# Autodesk Inventor assembly: Arm
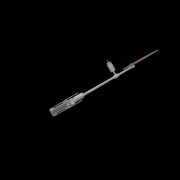
[picture p0: Inventor's stored thumbnail of the model, 180x180]
Saved by Autodesk Inventor 2020 (Build 240168000, 168)
## iProperties
Created: 2020-03-24
Part Number: Arm
Document SubType Name: Assembly
Designer: valer
Mass: 4853.44 g
Surface Area: 23913.7 cm^2
Volume: 23972.4 cm^3
Density: 0.202459 g/cm^3
Author: valer
## Documents named in this file (17)
- C:\Users\valer\Desktop\drummingrobot\src\Arm.iam
- C:\Users\valer\Desktop\drummingrobot\src\UpperArm.ipt
- C:\Users\valer\Desktop\drummingrobot\src\UpperArmBracket.ipt
- C:\Users\valer\Desktop\drummingrobot\src\Forearm.ipt
- C:\Users\valer\Desktop\drummingrobot\src\external\Drumstick.ipt
- C:\Users\valer\Desktop\drummingrobot\src\external\ForearmShaftCollar.ipt
- C:\Users\valer\Desktop\drummingrobot\src\external\PushSolenoid.ipt
- C:\Users\valer\Desktop\drummingrobot\src\external\UpperArmActuatorBody.ipt
- C:\Users\valer\Desktop\drummingrobot\src\external\UpperArmActuatorShaft.ipt
- C:\Users\valer\Desktop\drummingrobot\src\external\ForearmActuatorBody.ipt
- C:\Users\valer\Desktop\drummingrobot\src\external\ForearmActuatorShaft.ipt
- C:\Users\valer\Desktop\drummingrobot\src\external\Drums.ipt
- C:\Users\valer\Desktop\drummingrobot\src\ForearmActuatorConnector.ipt
- C:\Users\valer\Desktop\drummingrobot\src\UpperArmBracketMirror.ipt
- C:\Users\valer\Desktop\drummingrobot\src\UpperArmActuatorBracket.ipt
- C:\Users\valer\Desktop\drummingrobot\src\UpperArmActuatorBracketMirror.ipt
- C:\Users\valer\Desktop\drummingrobot\src\UpperArmMount.ipt
## Components (17 placed, 15 different names)
1. Drumstick:1 — Mate:79, Flush:3
2. ShaftCollar1/2:1 — Mate:79, Flush:3, Mate:236, Flush:18
3. PushSolenoid:1 — Mate:258, Mate:259
4. FA-35-S-12-1:1 — Mate:257, Mate:266
5. Forearm:1 — Flush:17, Mate:227, Mate:236, Flush:18, Mate:239, Mate:244, Mate:258, Mate:259
6. FA-35-S-12-1:2 — Mate:238, Flush:20, Mate:266
7. ForearmActuatorBody:1 — Mate:231, Mate:232, Mate:234, Flush:19
8. Drums:1 — Flush:13
9. ForearmActuatorShaft:3 — Flush:17, Mate:231, Mate:232, Mate:241, Mate:243, Angle:10, Mate:246
10. UpperArm:3 — Mate:227, Mate:234, Mate:238, Flush:19, Flush:20, Mate:248, Mate:249, Mate:263, Mate:264, Mate:265
11. ForearmActuatorConnector:1 — Mate:239, Mate:241, Mate:245, Angle:10, Mate:246
12. ForearmActuatorConnector:2 — Mate:243, Mate:244, Mate:245
13. UpperArmBracket:5 — Mate:249, Mate:254, Mate:255, Mate:256, Flush:21, Mate:265, Mate:267, Mate:272
14. UpperArmBracketMirror:1 — Mate:248, Mate:251, Mate:252, Mate:253, Flush:21, Mate:263, Mate:264, Mate:270, Mate:271
15. UpperArmActuatorBracket:1 — Mate:254, Mate:255, Mate:256, Mate:262
16. UpperArmActuatorBracketMirror:1 — Mate:251, Mate:252, Mate:253, Mate:257
17. UpperArmMount:1 — Mate:267, Mate:270, Mate:271, Mate:272, Mate:273
## Relationships (42: Mate 34, Flush 7, Angle 1)
- Mate:79: Drumstick:1 ↔ ShaftCollar1/2:1
- Flush:3 (304.8 mm): Drumstick:1 ↔ ShaftCollar1/2:1
- Flush:13 (508 mm): Drums:1
- Flush:17: Forearm:1 ↔ ForearmActuatorShaft:3
- Mate:227: Forearm:1 ↔ UpperArm:3
- Mate:231: ForearmActuatorBody:1 ↔ ForearmActuatorShaft:3
- Mate:232: ForearmActuatorBody:1 ↔ ForearmActuatorShaft:3
- Mate:234: ForearmActuatorBody:1 ↔ UpperArm:3
- Mate:236: ShaftCollar1/2:1 ↔ Forearm:1
- Flush:18 (12.7 mm): ShaftCollar1/2:1 ↔ Forearm:1
- Mate:238: FA-35-S-12-1:2 ↔ UpperArm:3
- Flush:19: ForearmActuatorBody:1 ↔ UpperArm:3
- Flush:20: FA-35-S-12-1:2 ↔ UpperArm:3
- Mate:239: Forearm:1 ↔ ForearmActuatorConnector:1
- Mate:241: ForearmActuatorShaft:3 ↔ ForearmActuatorConnector:1
- Mate:243: ForearmActuatorShaft:3 ↔ ForearmActuatorConnector:2
- Mate:244: Forearm:1 ↔ ForearmActuatorConnector:2
- Mate:245: ForearmActuatorConnector:1 ↔ ForearmActuatorConnector:2
- Angle:10 (-180 deg): ForearmActuatorShaft:3 ↔ ForearmActuatorConnector:1
- Mate:246: ForearmActuatorShaft:3 ↔ ForearmActuatorConnector:1
- Mate:248: UpperArm:3 ↔ UpperArmBracketMirror:1
- Mate:249: UpperArm:3 ↔ UpperArmBracket:5
- Mate:251: UpperArmBracketMirror:1 ↔ UpperArmActuatorBracketMirror:1
- Mate:252: UpperArmBracketMirror:1 ↔ UpperArmActuatorBracketMirror:1
- Mate:253: UpperArmBracketMirror:1 ↔ UpperArmActuatorBracketMirror:1
- Mate:254: UpperArmBracket:5 ↔ UpperArmActuatorBracket:1
- Mate:255: UpperArmBracket:5 ↔ UpperArmActuatorBracket:1
- Mate:256: UpperArmBracket:5 ↔ UpperArmActuatorBracket:1
- Flush:21: UpperArmBracket:5 ↔ UpperArmBracketMirror:1
- Mate:257: FA-35-S-12-1:1 ↔ UpperArmActuatorBracketMirror:1
- Mate:258: PushSolenoid:1 ↔ Forearm:1
- Mate:259: PushSolenoid:1 ↔ Forearm:1
- Mate:262: UpperArmActuatorBracket:1
- Mate:263: UpperArm:3 ↔ UpperArmBracketMirror:1
- Mate:264: UpperArm:3 ↔ UpperArmBracketMirror:1
- Mate:265: UpperArm:3 ↔ UpperArmBracket:5
- Mate:266: FA-35-S-12-1:1 ↔ FA-35-S-12-1:2
- Mate:267: UpperArmBracket:5 ↔ UpperArmMount:1
- Mate:270: UpperArmBracketMirror:1 ↔ UpperArmMount:1
- Mate:271: UpperArmBracketMirror:1 ↔ UpperArmMount:1
- Mate:272: UpperArmBracket:5 ↔ UpperArmMount:1
- Mate:273: UpperArmMount:1
